# Autodesk Inventor assembly: Anderson3x5block
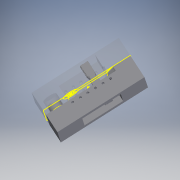
[picture p0: Inventor's stored thumbnail of the model, 180x180]
Saved by Autodesk Inventor 2018 (Build 220112000, 112)
## iProperties
Created: 2017-09-08
Part Number: Anderson3x5block
Document SubType Name: Assembly
Designer: Srinity
Author: Srinity
## Documents named in this file (4)
- C:\Users\Srinity\Documents\DIY Projects\ModularFRCPlatform\Anderson3x5block.iam
- C:\Users\Srinity\Documents\DIY Projects\ModularFRCPlatform\AndersonA.ipt
- C:\Users\Srinity\Documents\DIY Projects\ModularFRCPlatform\AndersonA_MIR.ipt
- C:\Users\Srinity\Documents\DIY Projects\ModularFRCPlatform\AndersonPP.ipt
## Components (4 placed, 3 different names)
1. AndersonA:1 — Mate:1, Flush:1, Flush:2, Mate:3, Mate:4, Angle:1
2. AndersonA_MIR:1 — Mate:1, Flush:1, Flush:2, Mate:5, Mate:6
3. AndersonPP:1 — Mate:3, Mate:4, Angle:1
4. AndersonPP:2 — Mate:5, Mate:6
## Relationships (8: Mate 5, Flush 2, Angle 1)
- Mate:1: AndersonA:1 ↔ AndersonA_MIR:1
- Flush:1: AndersonA:1 ↔ AndersonA_MIR:1
- Flush:2: AndersonA:1 ↔ AndersonA_MIR:1
- Mate:3: AndersonA:1 ↔ AndersonPP:1
- Mate:4: AndersonA:1 ↔ AndersonPP:1
- Angle:1 (0 deg): AndersonA:1 ↔ AndersonPP:1
- Mate:5: AndersonA_MIR:1 ↔ AndersonPP:2
- Mate:6: AndersonA_MIR:1 ↔ AndersonPP:2
